# Autodesk Inventor assembly: AXp3c test assembly
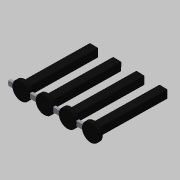
[picture p0: Inventor's stored thumbnail of the model, 180x180]
Saved by Autodesk Inventor 2019.3 (Build 233278000, 278)
## iProperties
Created: 2019-02-28
Part Number: AXp3c test assembly
Document SubType Name: Assembly
Designer: Varga Daniel
Author: Varga Daniel
## Documents named in this file (7)
- C:\!_Dani\!_cloud\OneDrive\!_munka\Revolution\RevvyDemoKit\Structural parts\RFQ\SLS print collection Rev 1\AXp3c\AXp3c test assembly.iam
- C:\!_Dani\!_cloud\OneDrive\!_munka\Revolution\RevvyDemoKit\Structural parts\RFQ\SLS print collection Rev 1\AXp3c\AXp3c_3,60.ipt
- C:\!_Dani\!_cloud\OneDrive\!_munka\Revolution\RevvyDemoKit\Structural parts\RFQ\SLS print collection Rev 1\AXp3c.ipt
- C:\!_Dani\!_cloud\OneDrive\!_munka\Revolution\RevvyDemoKit\Structural parts\RFQ\SLS print collection Rev 1\AXp3c\AXp3c_3,65.ipt
- C:\!_Dani\!_cloud\OneDrive\!_munka\Revolution\RevvyDemoKit\Structural parts\RFQ\SLS print collection Rev 1\AXp3c\AXp3c_3,70.ipt
- C:\!_Dani\!_cloud\OneDrive\!_munka\Revolution\RevvyDemoKit\Structural parts\RFQ\SLS print collection Rev 1\AXp3c\AXp3c_3,75.ipt
- C:\!_Dani\!_cloud\OneDrive\!_munka\Revolution\RevvyDemoKit\Structural parts\RFQ\SLS print collection Rev 1\AXp3c\pin_interconnect_3.ipt
## Components (5 placed, 5 different names)
1. AXp3c_3,75:4 — Tangent:4, Flush:2, Flush:3, Flush:4, Flush:7, Mate:1
2. AXp3c_3,70:3 — Tangent:3, Flush:1, Flush:4, Flush:5
3. AXp3c_3,65:2 — Tangent:2, Flush:1, Flush:2, Flush:5, Flush:6
4. AXp3c_3,60:1 — Tangent:1, Flush:3, Flush:6
5. pin_interconnect_3:1 — Flush:7, Mate:1, Angle:1
## Relationships (13: Flush 7, Tangent 4, Mate 1, Angle 1)
- Tangent:1: AXp3c_3,60:1
- Tangent:2: AXp3c_3,65:2
- Tangent:3: AXp3c_3,70:3
- Tangent:4: AXp3c_3,75:4
- Flush:1: AXp3c_3,70:3 ↔ AXp3c_3,65:2
- Flush:2: AXp3c_3,75:4 ↔ AXp3c_3,65:2
- Flush:3: AXp3c_3,75:4 ↔ AXp3c_3,60:1
- Flush:4 (10 mm): AXp3c_3,75:4 ↔ AXp3c_3,70:3
- Flush:5 (10 mm): AXp3c_3,70:3 ↔ AXp3c_3,65:2
- Flush:6 (10 mm): AXp3c_3,65:2 ↔ AXp3c_3,60:1
- Flush:7 (0.3 mm): AXp3c_3,75:4 ↔ pin_interconnect_3:1
- Mate:1: AXp3c_3,75:4 ↔ pin_interconnect_3:1
- Angle:1 (0 deg): pin_interconnect_3:1
